# Autodesk Inventor assembly: 0304_練習3
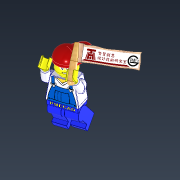
[picture p0: Inventor's stored thumbnail of the model, 180x180]
Saved by Autodesk Inventor 2022 (Build 260153000, 153)
## iProperties
Created: 2022-03-04
Part Number: 0304_練習3
Document SubType Name: Assembly
Designer: user
Author: user
## Documents named in this file (7)
- D:\pomelo\大一\下學期\機械設計製圖\PME1017_110033226\0304_練習3.iam
- D:\pomelo\大一\下學期\機械設計製圖\PME1017_110033226\0304_練習.iam
- D:\pomelo\大一\下學期\機械設計製圖\PME1017_110033226\0304_練習2.iam
- D:\pomelo\大一\下學期\機械設計製圖\教材_LEGOmini_2022_20220218\X02598_LEGOmini_Hat_R.ipt
- D:\pomelo\大一\下學期\機械設計製圖\教材_LEGOmini_2022_20220218\X02598_LEGOmini_Head_Y.ipt
- D:\pomelo\大一\下學期\機械設計製圖\教材_LEGOmini_2022_20220218\X02598_LEGOmini_PMECAD_LEGOmini_Flag.ipt
- D:\pomelo\大一\下學期\機械設計製圖\教材_LEGOmini_2022_20220218\X02598_LEGOmini_PMECAD_LEGOmini_FlagFrame.ipt
## Components (6 placed, 6 different names)
1. 0304_練習:1 [sub-assembly] — 貼合:3, 貼合:14
2. 0304_練習2:1 [sub-assembly] — 貼合:1, 貼合:3, 貼合:4, 角度:1, 對稱:1, 貼合:7, 貼合:8, 貼合:11, 貼合:14, 貼合:16, 角度:2, 齊平:1, 貼合:17
3. X02598_LEGOmini_Hat_R:1 — 貼合:5, 貼合:6
4. X02598_LEGOmini_Head_Y:1 — 貼合:5, 貼合:6, 貼合:7, 貼合:8
5. X02598_LEGOmini_PMECAD_LEGOmini_Flag:1 — 貼合:12, 貼合:13, 貼合:15
6. X02598_LEGOmini_PMECAD_LEGOmini_FlagFrame:1 — 貼合:11, 貼合:12, 貼合:13, 貼合:15, 貼合:17
## Relationships (18: Mate 14, Angle 2, Symmetry 1, Flush 1)
- 貼合:1 [Mate]: 0304_練習2:1
- 貼合:3 [Mate]: 0304_練習:1 ↔ 0304_練習2:1
- 貼合:4 [Mate]: 0304_練習2:1
- 角度:1 [Angle] (0 deg): 0304_練習2:1
- 對稱:1 [Symmetry]: 0304_練習2:1
- 貼合:5 [Mate]: X02598_LEGOmini_Hat_R:1 ↔ X02598_LEGOmini_Head_Y:1
- 貼合:6 [Mate]: X02598_LEGOmini_Hat_R:1 ↔ X02598_LEGOmini_Head_Y:1
- 貼合:7 [Mate]: 0304_練習2:1 ↔ X02598_LEGOmini_Head_Y:1
- 貼合:8 [Mate]: 0304_練習2:1 ↔ X02598_LEGOmini_Head_Y:1
- 貼合:11 [Mate]: 0304_練習2:1 ↔ X02598_LEGOmini_PMECAD_LEGOmini_FlagFrame:1
- 貼合:12 [Mate]: X02598_LEGOmini_PMECAD_LEGOmini_Flag:1 ↔ X02598_LEGOmini_PMECAD_LEGOmini_FlagFrame:1
- 貼合:13 [Mate]: X02598_LEGOmini_PMECAD_LEGOmini_Flag:1 ↔ X02598_LEGOmini_PMECAD_LEGOmini_FlagFrame:1
- 貼合:14 [Mate]: 0304_練習:1 ↔ 0304_練習2:1
- 貼合:15 [Mate]: X02598_LEGOmini_PMECAD_LEGOmini_Flag:1 ↔ X02598_LEGOmini_PMECAD_LEGOmini_FlagFrame:1
- 貼合:16 [Mate]: 0304_練習2:1
- 角度:2 [Angle] (0 deg): 0304_練習2:1
- 齊平:1 [Flush] (-4 mm): 0304_練習2:1
- 貼合:17 [Mate]: 0304_練習2:1 ↔ X02598_LEGOmini_PMECAD_LEGOmini_FlagFrame:1
